# Autodesk Inventor assembly: box
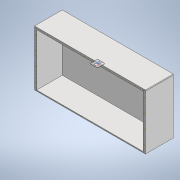
[picture p0: Inventor's stored thumbnail of the model, 180x180]
Saved by Autodesk Inventor 2021 (Build 250183000, 183)
## iProperties
Created: 2021-03-15
Part Number: box
Document SubType Name: Assembly
Designer: kanyk
Author: kanyk
## Documents named in this file (3)
- D:\Project\AllTaskFromTUL\TUL\20202021\ZKO\box.iam
- D:\Project\AllTaskFromTUL\TUL\20202021\ZKO\bottom.ipt
- D:\Project\AllTaskFromTUL\TUL\20202021\ZKO\top.ipt
## Components (2 placed, 2 different names)
1. bottom:1 — Stejný směr:1
2. top:1 — Stejný směr:1
## Relationships (1: Flush 1)
- Stejný směr:1 [Flush]: bottom:1 ↔ top:1
